# Autodesk Inventor assembly: ASY ДМФ лоток 040 илоотвод
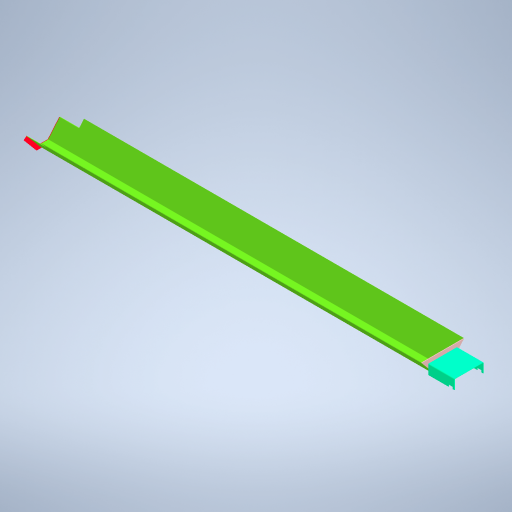
[picture p0: Inventor's stored thumbnail of the model, 512x512]
Saved by Autodesk Inventor 2024.2 (Build 282272000, 272)
## iProperties
Created: 2024-05-14
Part Number: ASY ДМФ лоток 040 илоотвод
Document SubType Name: Assembly
Designer: admin
Author: admin
## Documents named in this file (5)
- C:\Users\admin\YandexDisk-badmisterfox\домашниий пк\Inventor\DMF-Disk-Micro-Filter\ASY ДМФ лоток 040 илоотвод.iam
- C:\Users\admin\YandexDisk-badmisterfox\домашниий пк\Inventor\DMF-Disk-Micro-Filter\ДМС 040 лоток илоотвод.ipt
- C:\Users\admin\YandexDisk-badmisterfox\домашниий пк\Inventor\DMF-Disk-Micro-Filter\ДМС 304 торец лотка кормовой.ipt
- C:\Users\admin\YandexDisk-badmisterfox\домашниий пк\Inventor\DMF-Disk-Micro-Filter\ДМС 310 швеллер лотка.ipt
- C:\Users\admin\YandexDisk-badmisterfox\домашниий пк\Inventor\DMF-Disk-Micro-Filter\ДМФ 044 фланец лотка.ipt
## Components (4 placed, 4 different names)
1. ДМС 040 лоток илоотвод:1
2. ДМС 304 торец лотка кормовой:1 — Flush:1, Mate:1
3. ДМС 310 швеллер лотка:1 — Flush:1, Mate:1, Flush:2
4. ДМФ 044 фланец лотка:1
## Relationships (5: WeldJoint 2, Flush 2, Mate 1)
- [WeldJoint]: ДМС 040 лоток илоотвод:1 ↔ ДМС 304 торец лотка кормовой:1
- [WeldJoint]: ДМС 040 лоток илоотвод:1 ↔ ДМФ 044 фланец лотка:1
- Flush:1 (20 mm): ДМС 304 торец лотка кормовой:1 ↔ ДМС 310 швеллер лотка:1
- Mate:1: ДМС 304 торец лотка кормовой:1 ↔ ДМС 310 швеллер лотка:1
- Flush:2: ДМС 310 швеллер лотка:1
